# Autodesk Inventor assembly: l12_50mm_in
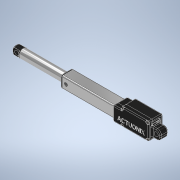
[picture p0: Inventor's stored thumbnail of the model, 180x180]
Saved by Autodesk Inventor 2021 (Build 250183000, 183)
## iProperties
Created: 2016-10-05
Part Number: l12_50mm_in
Document SubType Name: Assembly
Designer: Kafuko Martha
Sending System: PRO/ENGINEER BY PARAMETRIC TECHNOLOGY CORPORATION, 2004440
Preprocessor: PRO/ENGINEER BY PARAMETRIC TECHNOLOGY CORPORATION, 2004440
Title: L12_50MM_ASM
Author: Mike
Revision Number: 1LAST_VERSION
## Documents named in this file (10)
- C:\Users\Work\Desktop\Modified Mounting Bracket\_ToSend\#Linear Actuator\Linear Actuator.iam
- C:\Users\Work\Desktop\Modified Mounting Bracket\_ToSend\#Linear Actuator\EXTENSION_10404_50MM.ipt
- C:\Users\Work\Desktop\Modified Mounting Bracket\_ToSend\#Linear Actuator\CLAMSHELL_BOT_10417.ipt
- C:\Users\Work\Desktop\Modified Mounting Bracket\_ToSend\#Linear Actuator\CLAMSHELL_TOP_10416.ipt
- C:\Users\Work\Desktop\Modified Mounting Bracket\_ToSend\#Linear Actuator\FASTENER_10427.ipt
- C:\Users\Work\Desktop\Modified Mounting Bracket\_ToSend\#Linear Actuator\GUIDE_10429.ipt
- C:\Users\Work\Desktop\Modified Mounting Bracket\_ToSend\#Linear Actuator\NUT_10419.ipt
- C:\Users\Work\Desktop\Modified Mounting Bracket\_ToSend\#Linear Actuator\SHAFT_10409_50MM.ipt
- C:\Users\Work\Desktop\Modified Mounting Bracket\_ToSend\#Linear Actuator\PLUG_10428.ipt
- C:\Users\Work\Desktop\Modified Mounting Bracket\_ToSend\#Linear Actuator\GROMMET_3_HOLE.ipt
## Components (12 placed, 12 different names)
1. EXTENSION_10404_50MM_74 — Mate:18, Mate:19, Mate:20, Mate:23, Angle:7, Flush:2, Angle:8
2. CLAMSHELL_BOT_10417_75 — Mate:1, Mate:2, Mate:3, Mate:4, Angle:1, Angle:2, Angle:3, Angle:4, Mate:5, Mate:6, Mate:7, Mate:8, Mate:9, Flush:1, Mate:15, Angle:5, Mate:18, Mate:19, Mate:20, Angle:6, Mate:26
3. CLAMSHELL_TOP_10416_76 — Mate:7, Mate:8, Mate:9, Mate:10, Mate:11, Mate:12, Mate:13
4. FASTENER_10427_77 — Mate:1, Angle:4, Mate:13
5. FASTENER_10427_78 — Mate:4, Angle:1, Mate:12
6. FASTENER_10427_79 — Mate:3, Angle:2, Mate:11
7. FASTENER_10427_80 — Mate:2, Angle:3, Mate:10
8. GUIDE_10429_81 — Mate:23, Angle:7, Flush:2
9. NUT_10419_82 — Mate:15, Angle:5, Mate:21, Mate:22, Mate:26
10. SHAFT_10409_50MM_83 — Mate:21, Mate:22, Angle:6, Mate:24, Mate:25
11. PLUG_10428_84 — Mate:24, Mate:25, Angle:8
12. GROMMET_3_HOLE_85 — Mate:5, Mate:6, Flush:1
## Relationships (33: Mate 23, Angle 8, Flush 2)
- Mate:1: CLAMSHELL_BOT_10417_75 ↔ FASTENER_10427_77
- Mate:2: CLAMSHELL_BOT_10417_75 ↔ FASTENER_10427_80
- Mate:3: CLAMSHELL_BOT_10417_75 ↔ FASTENER_10427_79
- Mate:4: CLAMSHELL_BOT_10417_75 ↔ FASTENER_10427_78
- Angle:1 (0 deg): CLAMSHELL_BOT_10417_75 ↔ FASTENER_10427_78
- Angle:2 (0 deg): CLAMSHELL_BOT_10417_75 ↔ FASTENER_10427_79
- Angle:3 (0 deg): CLAMSHELL_BOT_10417_75 ↔ FASTENER_10427_80
- Angle:4 (0 deg): CLAMSHELL_BOT_10417_75 ↔ FASTENER_10427_77
- Mate:5 (0.25 mm): CLAMSHELL_BOT_10417_75 ↔ GROMMET_3_HOLE_85
- Mate:6: CLAMSHELL_BOT_10417_75 ↔ GROMMET_3_HOLE_85
- Mate:7: CLAMSHELL_BOT_10417_75 ↔ CLAMSHELL_TOP_10416_76
- Mate:8: CLAMSHELL_BOT_10417_75 ↔ CLAMSHELL_TOP_10416_76
- Mate:9: CLAMSHELL_BOT_10417_75 ↔ CLAMSHELL_TOP_10416_76
- Mate:10: CLAMSHELL_TOP_10416_76 ↔ FASTENER_10427_80
- Mate:11: CLAMSHELL_TOP_10416_76 ↔ FASTENER_10427_79
- Mate:12: CLAMSHELL_TOP_10416_76 ↔ FASTENER_10427_78
- Mate:13: CLAMSHELL_TOP_10416_76 ↔ FASTENER_10427_77
- Flush:1 (0.936 mm): CLAMSHELL_BOT_10417_75 ↔ GROMMET_3_HOLE_85
- Mate:15: CLAMSHELL_BOT_10417_75 ↔ NUT_10419_82
- Angle:5 (270 deg): CLAMSHELL_BOT_10417_75 ↔ NUT_10419_82
- Mate:18: EXTENSION_10404_50MM_74 ↔ CLAMSHELL_BOT_10417_75
- Mate:19: EXTENSION_10404_50MM_74 ↔ CLAMSHELL_BOT_10417_75
- Mate:20: EXTENSION_10404_50MM_74 ↔ CLAMSHELL_BOT_10417_75
- Mate:21: NUT_10419_82 ↔ SHAFT_10409_50MM_83
- Mate:22: NUT_10419_82 ↔ SHAFT_10409_50MM_83
- Angle:6 (0 deg): CLAMSHELL_BOT_10417_75 ↔ SHAFT_10409_50MM_83
- Mate:23: EXTENSION_10404_50MM_74 ↔ GUIDE_10429_81
- Angle:7 (0 deg): EXTENSION_10404_50MM_74 ↔ GUIDE_10429_81
- Flush:2: EXTENSION_10404_50MM_74 ↔ GUIDE_10429_81
- Mate:24: SHAFT_10409_50MM_83 ↔ PLUG_10428_84
- Mate:25: SHAFT_10409_50MM_83 ↔ PLUG_10428_84
- Mate:26: CLAMSHELL_BOT_10417_75 ↔ NUT_10419_82
- Angle:8 (0 deg): EXTENSION_10404_50MM_74 ↔ PLUG_10428_84
